# Autodesk Inventor assembly: Right Internal Side Panel Assembly
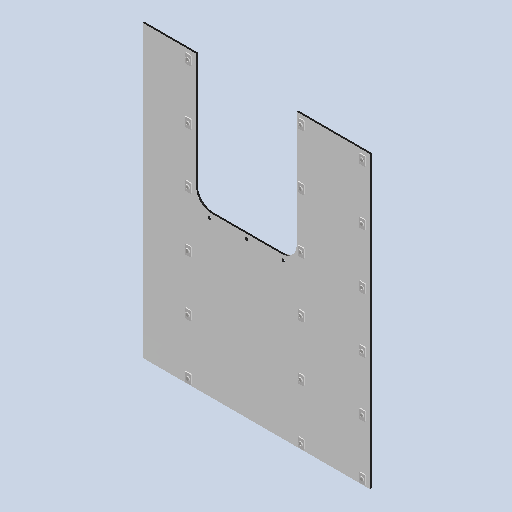
[picture p0: Inventor's stored thumbnail of the model, 512x512]
Saved by Autodesk Inventor 2024 (Build 280153000, 153)
## iProperties
Created: 2024-10-26
Part Number: Right Internal Side Panel Assembly
Document SubType Name: Assembly
Designer: Ishaan
Author: Ishaan
## Documents named in this file (4)
- E:\Projects\Axiom--IDEX-3D-Printer\CAD\08 - Side Panelling\Right Internal Side Panel Assembly.iam
- E:\Projects\Axiom--IDEX-3D-Printer\CAD\08 - Side Panelling\Side Internal Side Panel R2.ipt
- E:\Projects\Axiom--IDEX-3D-Printer\CAD\00 - COTS Components\Hardware\Low Profile M5x8.ipt
- E:\Projects\Axiom--IDEX-3D-Printer\CAD\00 - COTS Components\Hardware\M5 T SLOT NUT.ipt
## Components (37 placed, 3 different names)
1. Side Internal Side Panel R2:1 — Insert:1, Insert:2, Insert:3, Insert:4, Insert:5, Insert:6, Angle:1, Angle:2, Angle:3
2. Low Profile M5x8:1 — Insert:1
3. Low Profile M5x8:2 — Insert:2
4. Low Profile M5x8:3 — Insert:3
5. Low Profile M5x8:4
6. Low Profile M5x8:5
7. Low Profile M5x8:6
8. Low Profile M5x8:7
9. Low Profile M5x8:8
10. Low Profile M5x8:9
11. Low Profile M5x8:10
12. Low Profile M5x8:11
13. Low Profile M5x8:12
14. Low Profile M5x8:13
15. Low Profile M5x8:14
16. Low Profile M5x8:15
17. Low Profile M5x8:16
18. Low Profile M5x8:17
19. Low Profile M5x8:18
20. M5 T SLOT NUT:1 — Insert:4, Angle:3
21. M5 T SLOT NUT:2 — Insert:5, Angle:2
22. M5 T SLOT NUT:3 — Insert:6, Angle:1
23. M5 T SLOT NUT:4
24. M5 T SLOT NUT:5
25. M5 T SLOT NUT:6
26. M5 T SLOT NUT:7
27. M5 T SLOT NUT:8
28. M5 T SLOT NUT:9
29. M5 T SLOT NUT:10
30. M5 T SLOT NUT:11
31. M5 T SLOT NUT:12
32. M5 T SLOT NUT:13
33. M5 T SLOT NUT:14
34. M5 T SLOT NUT:15
35. M5 T SLOT NUT:16
36. M5 T SLOT NUT:17
37. M5 T SLOT NUT:18
## Component patterns: (6 elements, first: Low Profile M5x8:1 + Low Profile M5x8:2 + Low Profile M5x8:3), (6 elements, first: M5 T SLOT NUT:1 + M5 T SLOT NUT:2 + M5 T SLOT NUT:3)
## Relationships (9: Insert 6, Angle 3)
- Insert:1: Side Internal Side Panel R2:1 ↔ Low Profile M5x8:1
- Insert:2: Side Internal Side Panel R2:1 ↔ Low Profile M5x8:2
- Insert:3: Side Internal Side Panel R2:1 ↔ Low Profile M5x8:3
- Insert:4 (2 mm): Side Internal Side Panel R2:1 ↔ M5 T SLOT NUT:1
- Insert:5 (2 mm): Side Internal Side Panel R2:1 ↔ M5 T SLOT NUT:2
- Insert:6 (2 mm): Side Internal Side Panel R2:1 ↔ M5 T SLOT NUT:3
- Angle:1 (0 deg): Side Internal Side Panel R2:1 ↔ M5 T SLOT NUT:3
- Angle:2 (0 deg): Side Internal Side Panel R2:1 ↔ M5 T SLOT NUT:2
- Angle:3 (0 deg): Side Internal Side Panel R2:1 ↔ M5 T SLOT NUT:1
